# Autodesk Inventor assembly: OrangePICover
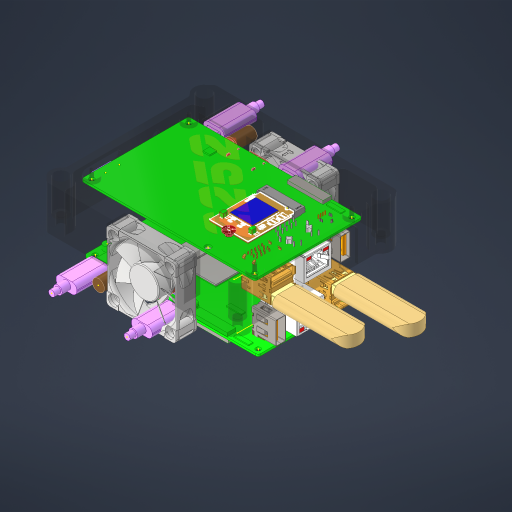
[picture p0: Inventor's stored thumbnail of the model, 512x512]
Saved by Autodesk Inventor 2023 (Build 270158000, 158)
## iProperties
Created: 2024-02-19
Part Number: OrangePICover
Document SubType Name: Assembly
Designer: Paul
Author: Paul
## Documents named in this file (5)
- C:\Users\dlangdon\Documents\GitHub\Crescendo_2024-CAD\2024 Robot\COMMON PARTS\ELECTRONICS\OrangePi\Orange_Pi_Cover_001\OrangePICover.iam
- C:\Users\dlangdon\Documents\GitHub\Crescendo_2024-CAD\2024 Robot\COMMON PARTS\ELECTRONICS\OrangePi\Orange_Pi_Cover_001\orange pi\OPi5_pcb_asm-0809.iam
- C:\Users\dlangdon\Documents\GitHub\Crescendo_2024-CAD\2024 Robot\COMMON PARTS\ELECTRONICS\OrangePi\Orange_Pi_Cover_001\orangepicover-001.ipt
- C:\Users\dlangdon\Documents\GitHub\Crescendo_2024-CAD\2024 Robot\COMMON PARTS\ELECTRONICS\OrangePi\Orange_Pi_Cover_001\noctua-NF-A4x10\Noctua-NF-A4x10.iam
- C:\Users\dlangdon\Documents\GitHub\Crescendo_2024-CAD\2024 Robot\COMMON PARTS\ELECTRONICS\OrangePi\Orange_Pi_Cover_001\orangepicover-001a.ipt
## Components (6 placed, 4 different names)
1. OPi5_pcb_asm-0809:1 [sub-assembly] — Flush:1, Flush:2, Insert:1, Insert:2
2. orangepicover-001:1 — Flush:1, Flush:2, Mate:6, Mate:8, Mate:9, Mate:11, Insert:1, Insert:2, Mate:12
3. orangepicover-001a:1
4. OPi5_pcb_asm-0809:2 [sub-assembly]
5. Noctua-NF-A4x10:1 [sub-assembly] — Mate:8, Mate:9, Mate:12
6. Noctua-NF-A4x10:2 [sub-assembly] — Mate:6, Mate:11
## Relationships (16: Mate 10, Flush 4, Insert 2)
- Flush:1: OPi5_pcb_asm-0809:1 ↔ orangepicover-001:1
- Flush:2: OPi5_pcb_asm-0809:1 ↔ orangepicover-001:1
- [Mate]: orangepicover-001:1 ↔ orangepicover-001a:1
- [Flush]: orangepicover-001:1 ↔ orangepicover-001a:1
- [Flush]: orangepicover-001:1 ↔ orangepicover-001a:1
- [Mate]: orangepicover-001a:1 ↔ OPi5_pcb_asm-0809:2
- [Mate]: orangepicover-001a:1 ↔ OPi5_pcb_asm-0809:2
- [Mate]: orangepicover-001a:1 ↔ OPi5_pcb_asm-0809:2
- [Mate]: orangepicover-001a:1 ↔ Noctua-NF-A4x10:2
- Mate:6: orangepicover-001:1 ↔ Noctua-NF-A4x10:2
- Mate:8: orangepicover-001:1 ↔ Noctua-NF-A4x10:1
- Mate:9: orangepicover-001:1 ↔ Noctua-NF-A4x10:1
- Mate:11: orangepicover-001:1 ↔ Noctua-NF-A4x10:2
- Insert:1: OPi5_pcb_asm-0809:1 ↔ orangepicover-001:1
- Insert:2: OPi5_pcb_asm-0809:1 ↔ orangepicover-001:1
- Mate:12: orangepicover-001:1 ↔ Noctua-NF-A4x10:1
